# Autodesk Inventor assembly: rapoukMiddleLegAssemblyv0
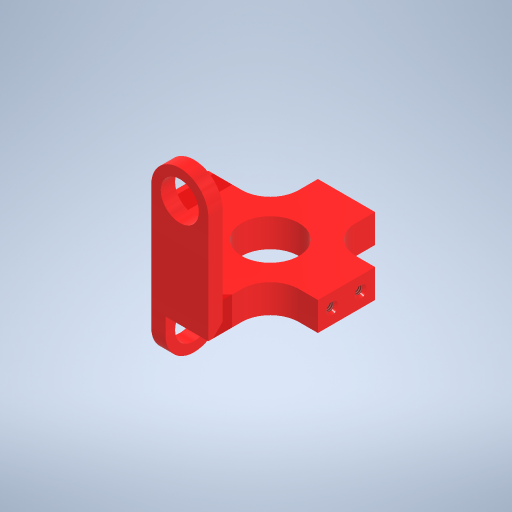
[picture p0: Inventor's stored thumbnail of the model, 512x512]
Saved by Autodesk Inventor 2024 (Build 280153000, 153)
## iProperties
Created: 2024-01-09
Part Number: rapoukMiddleLegAssemblyv0
Document SubType Name: Weldment
Designer: Roman Suk
Weld Material: Welded Aluminum-6061
Author: Roman Suk
## Documents named in this file (3)
- C:\Users\Roman Suk\Documents\Ročníkovka SŠ\CD\Technická dokumentace\rapoukMiddleLegAssemblyv0.iam
- C:\Users\Roman Suk\Documents\Ročníkovka SŠ\CD\Technická dokumentace\rapoukMiddleLeg0v3.ipt
- C:\Users\Roman Suk\Documents\Ročníkovka SŠ\CD\Technická dokumentace\rapoukMiddleLeg1v3.ipt
## Components (3 placed, 2 different names)
1. rapoukMiddleLeg0v3:1 — Mate:1, Flush:1, Flush:2, Mate:2, Flush:3, Flush:4
2. rapoukMiddleLeg1v3:1 — Mate:1, Flush:1, Flush:2
3. rapoukMiddleLeg1v3:2 — Mate:2, Flush:3, Flush:4
## Relationships (6: Flush 4, Mate 2)
- Mate:1: rapoukMiddleLeg0v3:1 ↔ rapoukMiddleLeg1v3:1
- Flush:1: rapoukMiddleLeg0v3:1 ↔ rapoukMiddleLeg1v3:1
- Flush:2: rapoukMiddleLeg0v3:1 ↔ rapoukMiddleLeg1v3:1
- Mate:2: rapoukMiddleLeg0v3:1 ↔ rapoukMiddleLeg1v3:2
- Flush:3: rapoukMiddleLeg0v3:1 ↔ rapoukMiddleLeg1v3:2
- Flush:4: rapoukMiddleLeg0v3:1 ↔ rapoukMiddleLeg1v3:2
